# Autodesk Inventor assembly: FinalBioprinter
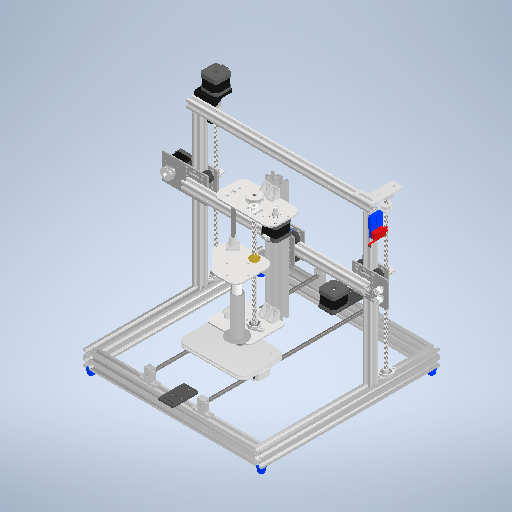
[picture p0: Inventor's stored thumbnail of the model, 512x512]
Saved by Autodesk Inventor 2025.2 (Build 292293000, 293)
## iProperties
Created: 2025-07-17
Part Number: FinalBioprinter
Document SubType Name: Assembly
Designer: Simon
Author: Simon
## Documents named in this file (51)
- C:\Users\Simon\Projects\Hydrogel-3D-Printer\Hardware\Bioprinter Machine Design\Final System\FinalBioprinter.iam
- C:\Users\Simon\Projects\Hydrogel-3D-Printer\Hardware\Bioprinter Machine Design\Final System\Final Gantry\2040_AluminimProfile_410.ipt
- C:\Users\Simon\Projects\Hydrogel-3D-Printer\Hardware\Bioprinter Machine Design\Final System\Final Gantry\2040_AluminimProfile_450.ipt
- C:\Users\Simon\Projects\Hydrogel-3D-Printer\Hardware\Bioprinter Machine Design\Final System\Final Gantry\2020_AluminiumProfile_380.ipt
- C:\Users\Simon\Projects\Hydrogel-3D-Printer\Hardware\Bioprinter Machine Design\Final System\Final Gantry\2020_AluminiumProfile_465.ipt
- C:\Users\Simon\Projects\Hydrogel-3D-Printer\Hardware\Bioprinter Machine Design\PartsFolder\bracket nema 17.ipt
- C:\Users\Simon\Projects\Hydrogel-3D-Printer\Hardware\Bioprinter Machine Design\PartsFolder\Pillow Block Bearing 1\Zinc Alloy Pillow Block Flange Bearing KFL08 ID-8mm.iam
- C:\Users\Simon\Projects\Hydrogel-3D-Printer\Hardware\Bioprinter Machine Design\PartsFolder\Stepper_17HS4401.ipt
- C:\Users\Simon\Projects\Hydrogel-3D-Printer\Hardware\Bioprinter Machine Design\PartsFolder\Flexible Coupling 5,8.ipt
- C:\Users\Simon\Projects\Hydrogel-3D-Printer\Hardware\Bioprinter Machine Design\Final System\Final Gantry\TR8x8-4_LeadScrew_385.ipt
- C:\Users\Simon\Projects\Hydrogel-3D-Printer\Hardware\Bioprinter Machine Design\PartsFolder\TR8x8-4_Nut.ipt
- C:\Users\Simon\Projects\Hydrogel-3D-Printer\Hardware\Bioprinter Machine Design\PartsFolder\Nema 17 Flat Mount.ipt
- C:\Users\Simon\Projects\Hydrogel-3D-Printer\Hardware\Bioprinter Machine Design\PartsFolder\GT2_20T_5.ipt
- C:\Users\Simon\Projects\Hydrogel-3D-Printer\Hardware\Bioprinter Machine Design\PartsFolder\SK8_LinearShaftSupport.ipt
- C:\Users\Simon\Projects\Hydrogel-3D-Printer\Hardware\Bioprinter Machine Design\Final System\Final Gantry\SteelShaft_444mm.ipt
- C:\Users\Simon\Projects\Hydrogel-3D-Printer\Hardware\Bioprinter Machine Design\PartsFolder\SC8UU\SC8UU.iam
- C:\Users\Simon\Projects\Hydrogel-3D-Printer\Hardware\Bioprinter Machine Design\PartsFolder\POM Wheel v2.ipt
- C:\Users\Simon\Projects\Hydrogel-3D-Printer\Hardware\Bioprinter Machine Design\PartsFolder\Carriage Plate v1.ipt
- C:\Users\Simon\Projects\Hydrogel-3D-Printer\Hardware\Bioprinter Machine Design\PartsFolder\Spacer v2.ipt
- C:\Users\Simon\Projects\Hydrogel-3D-Printer\Hardware\Bioprinter Machine Design\Final System\Final Gantry\2020_AluminiumProfile_460.ipt
- C:\Users\Simon\Projects\Hydrogel-3D-Printer\Hardware\Bioprinter Machine Design\Final System\Final Gantry\LeadCarriageConnector.ipt
- C:\Users\Simon\Projects\Hydrogel-3D-Printer\Hardware\Bioprinter Machine Design\Final System\Final Gantry\CarriagePlate_Motor.ipt
- C:\Users\Simon\Projects\Hydrogel-3D-Printer\Hardware\Bioprinter Machine Design\Final System\Final Gantry\CarriagePlate_Idler.ipt
- C:\Users\Simon\Projects\Hydrogel-3D-Printer\Hardware\Bioprinter Machine Design\PartsFolder\GT2_20T_Toothed_Idler_5.ipt
- C:\Users\Simon\Projects\Hydrogel-3D-Printer\Hardware\Bioprinter Machine Design\PartsFolder\Idler Pulley Plate.ipt
- C:\Users\Simon\Projects\Hydrogel-3D-Printer\Hardware\Bioprinter Machine Design\Final System\Final Gantry\BedHeatSink.ipt
- C:\Users\Simon\Projects\Hydrogel-3D-Printer\Hardware\Bioprinter Machine Design\PartsFolder\PeltierTEC1_12706.ipt
- C:\Users\Simon\Projects\Hydrogel-3D-Printer\Hardware\Bioprinter Machine Design\Final System\Final Gantry\ColdPlate.ipt
- C:\Users\Simon\Projects\Hydrogel-3D-Printer\Hardware\Bioprinter Machine Design\Final System\Final Gantry\LeadScrewEndMount.ipt
- C:\Users\Simon\Projects\Hydrogel-3D-Printer\Hardware\Bioprinter Machine Design\PartsFolder\GT2_36T_5.ipt
- C:\Users\Simon\Projects\Hydrogel-3D-Printer\Hardware\Bioprinter Machine Design\PartsFolder\GT2_30T_8.ipt
- C:\Users\Simon\Projects\Hydrogel-3D-Printer\Hardware\Bioprinter Machine Design\Gantry Concept 3\LimitSwitch.ipt
- C:\Users\Simon\Projects\Hydrogel-3D-Printer\Hardware\Bioprinter Machine Design\PartsFolder\Limit Switch\LimitSwitchPart.iam
- C:\Users\Simon\Projects\Hydrogel-3D-Printer\Hardware\Bioprinter Machine Design\Final System\Final Gantry\PrinterFeet.ipt
- C:\Users\Simon\Projects\Hydrogel-3D-Printer\Hardware\Bioprinter Machine Design\PartsFolder\0.4 nozzle.ipt
- C:\Users\Simon\Projects\Hydrogel-3D-Printer\Hardware\Bioprinter Machine Design\PartsFolder\E3D-v6 Heater Block for Sensor Cartridges.ipt
- C:\Users\Simon\Projects\Hydrogel-3D-Printer\Hardware\Bioprinter Machine Design\Final System\Final Extruder\TR8x8-4_LeadScrew_285.ipt
- C:\Users\Simon\Projects\Hydrogel-3D-Printer\Hardware\Bioprinter Machine Design\PartsFolder\GT2_16T_5.ipt
- C:\Users\Simon\Projects\Hydrogel-3D-Printer\Hardware\Bioprinter Machine Design\PartsFolder\GT2_48T_8.ipt
- C:\Users\Simon\Projects\Hydrogel-3D-Printer\Hardware\Bioprinter Machine Design\Final System\Final Extruder\2040_AluminimProfile_x.ipt
- C:\Users\Simon\Projects\Hydrogel-3D-Printer\Hardware\Bioprinter Machine Design\Final System\Final Extruder\Plunger.ipt
- C:\Users\Simon\Projects\Hydrogel-3D-Printer\Hardware\Bioprinter Machine Design\Final System\Final Extruder\CylinderAttachment.ipt
- C:\Users\Simon\Projects\Hydrogel-3D-Printer\Hardware\Bioprinter Machine Design\Final System\Final Extruder\SteelShaft_264.ipt
- C:\Users\Simon\Projects\Hydrogel-3D-Printer\Hardware\Bioprinter Machine Design\PartsFolder\SHF8.ipt
- C:\Users\Simon\Projects\Hydrogel-3D-Printer\Hardware\Bioprinter Machine Design\PartsFolder\LMK8UU.ipt
- C:\Users\Simon\Projects\Hydrogel-3D-Printer\Hardware\Bioprinter Machine Design\Final System\Final Extruder\TopMount.ipt
- C:\Users\Simon\Projects\Hydrogel-3D-Printer\Hardware\Bioprinter Machine Design\Final System\Final Extruder\MidMount.ipt
- C:\Users\Simon\Projects\Hydrogel-3D-Printer\Hardware\Bioprinter Machine Design\Final System\Final Extruder\BottomMount.ipt
- C:\Users\Simon\Projects\Hydrogel-3D-Printer\Hardware\Bioprinter Machine Design\PartsFolder\2020-corner-bracket.ipt
- C:\Users\Simon\Projects\Hydrogel-3D-Printer\Hardware\Bioprinter Machine Design\PartsFolder\GT2_20T_Smooth_Idler_5.ipt
- C:\Users\Simon\Projects\Hydrogel-3D-Printer\Hardware\Bioprinter Machine Design\Final System\Final Extruder\LoadCellMount.ipt
## Components (121 placed, 50 different names)
1. 2040_AluminimProfile_410:1 — Flush:67, Flush:68
2. 2040_AluminimProfile_450:1 — Flush:70, Mate:150
3. 2040_AluminimProfile_410:2 — Flush:70, Mate:151
4. 2040_AluminimProfile_450:2 — Flush:67, Flush:68, Flush:69
5. 2020_AluminiumProfile_380:1
6. 2020_AluminiumProfile_380:2
7. 2020_AluminiumProfile_465:1
8. bracket nema 17:1
9. Zinc Alloy Pillow Block Flange Bearing KFL08 ID-8mm:1 [sub-assembly]
10. Zinc Alloy Pillow Block Flange Bearing KFL08 ID-8mm:2 [sub-assembly]
11. Stepper_17HS4401:1
12. Flexible Coupling 5,8:1
13. TR8x8-4_LeadScrew_385:1
14. TR8x8-4_LeadScrew_385:2
15. TR8x8-4_Nut:1
16. TR8x8-4_Nut:2
17. Nema 17 Flat Mount:1 — Angle:11
18. Stepper_17HS4401:2 — Angle:11
19. GT2_20T_5:1
20. SK8_LinearShaftSupport:1
21. SK8_LinearShaftSupport:2
22. SK8_LinearShaftSupport:3
23. SK8_LinearShaftSupport:4 — Flush:69
24. SteelShaft_444mm:1
25. SteelShaft_444mm:2
26. SC8UU:1 [sub-assembly]
27. SC8UU:2 [sub-assembly]
28. POM Wheel v2:1
29. POM Wheel v2:2
30. POM Wheel v2:3
31. POM Wheel v2:4
32. Carriage Plate v1:1
33. Spacer v2:1
34. Spacer v2:2
35. Spacer v2:3
36. Spacer v2:4
37. Spacer v2:5
38. Spacer v2:6
39. Spacer v2:7
40. Spacer v2:8
41. POM Wheel v2:5
42. POM Wheel v2:6
43. POM Wheel v2:7
44. POM Wheel v2:8
45. Carriage Plate v1:2
46. Spacer v2:9
47. Spacer v2:10
48. Spacer v2:11
49. Spacer v2:12
50. Spacer v2:13
51. Spacer v2:14
52. Spacer v2:15
53. Spacer v2:16
54. 2020_AluminiumProfile_460:1
55. LeadCarriageConnector:1
56. LeadCarriageConnector:2
57. POM Wheel v2:9
58. POM Wheel v2:10
59. POM Wheel v2:11
60. POM Wheel v2:12
61. Carriage Plate v1:3
62. Spacer v2:17
63. Spacer v2:18
64. Spacer v2:19
65. Spacer v2:20
66. Spacer v2:21
67. Spacer v2:22
68. Spacer v2:23
69. Spacer v2:24
70. Carriage Plate v1:4 — Mate:202, Flush:82, Flush:83
71. Stepper_17HS4401:3
72. CarriagePlate_Motor:1
73. CarriagePlate_Idler:1
74. GT2_20T_Toothed_Idler_5:1
75. Spacer v2:25
76. Zinc Alloy Pillow Block Flange Bearing KFL08 ID-8mm:3 [sub-assembly]
77. Idler Pulley Plate:1
78. BedHeatSink:1
79. GT2_20T_Toothed_Idler_5:2
80. PeltierTEC1_12706:1
81. ColdPlate:1
82. Spacer v2:26
83. LeadScrewEndMount:1
84. GT2_20T_Toothed_Idler_5:3
85. Spacer v2:27
86. GT2_36T_5:1
87. GT2_30T_8:1
88. GT2_30T_8:2
89. LimitSwitch:1
90. LimitSwitch:2
91. LimitSwitchPart:1 [sub-assembly]
92. LimitSwitchPart:2 [sub-assembly]
93. PrinterFeet:1
94. PrinterFeet:2 — Mate:149
95. PrinterFeet:3
96. PrinterFeet:4
97. 0.4 nozzle:1
98. E3D-v6 Heater Block for Sensor Cartridges:1
99. TR8x8-4_LeadScrew_285:1
100. Stepper_17HS4401:4
101. TR8x8-4_Nut:3
102. GT2_16T_5:1
103. GT2_48T_8:1
104. Zinc Alloy Pillow Block Flange Bearing KFL08 ID-8mm:4 [sub-assembly]
105. 2040_AluminimProfile_x:1 — Mate:202, Flush:82, Flush:83
106. Plunger:1 — Mate:203
107. CylinderAttachment:1
108. Zinc Alloy Pillow Block Flange Bearing KFL08 ID-8mm:5 [sub-assembly]
109. SteelShaft_264:1
110. SHF8:1
111. SHF8:2
112. LMK8UU:1
113. TopMount:1
114. MidMount:1 — Mate:203
115. BottomMount:1
116. 2020-corner-bracket:1
117. 2020-corner-bracket:2
118. 2020-corner-bracket:3
119. 2020-corner-bracket:4
120. GT2_20T_Smooth_Idler_5:1
121. LoadCellMount:1
## Relationships (299: Mate 201, Flush 83, Angle 15)
- [Mate]: 2040_AluminimProfile_410:1 ↔ 2040_AluminimProfile_450:1
- [Flush]: 2040_AluminimProfile_410:1 ↔ 2040_AluminimProfile_450:1
- [Mate]: 2040_AluminimProfile_450:1 ↔ 2040_AluminimProfile_410:2
- [Flush]: 2040_AluminimProfile_450:1 ↔ 2040_AluminimProfile_410:2
- [Mate]: 2040_AluminimProfile_410:1 ↔ 2040_AluminimProfile_450:2
- [Mate]: 2040_AluminimProfile_450:1 ↔ 2020_AluminiumProfile_380:1
- [Mate]: 2040_AluminimProfile_450:2 ↔ 2020_AluminiumProfile_380:2
- [Flush]: 2040_AluminimProfile_450:1 ↔ 2020_AluminiumProfile_380:1
- [Flush]: 2040_AluminimProfile_450:2 ↔ 2020_AluminiumProfile_380:2
- [Mate]: 2020_AluminiumProfile_380:2 ↔ 2020_AluminiumProfile_465:1
- [Flush]: 2020_AluminiumProfile_380:2 ↔ 2020_AluminiumProfile_465:1
- [Flush]: 2020_AluminiumProfile_380:2 ↔ 2020_AluminiumProfile_465:1
- [Flush]: 2020_AluminiumProfile_380:1 ↔ 2020_AluminiumProfile_465:1
- [Mate]: 2040_AluminimProfile_450:1 ↔ Zinc Alloy Pillow Block Flange Bearing KFL08 ID-8mm:1
- [Mate]: 2040_AluminimProfile_450:2 ↔ Zinc Alloy Pillow Block Flange Bearing KFL08 ID-8mm:2
- [Mate]: 2040_AluminimProfile_450:1 ↔ Zinc Alloy Pillow Block Flange Bearing KFL08 ID-8mm:1
- [Mate]: 2040_AluminimProfile_450:2 ↔ Zinc Alloy Pillow Block Flange Bearing KFL08 ID-8mm:2
- [Flush]: Zinc Alloy Pillow Block Flange Bearing KFL08 ID-8mm:1 ↔ Zinc Alloy Pillow Block Flange Bearing KFL08 ID-8mm:2
- [Mate]: 2020_AluminiumProfile_465:1 ↔ bracket nema 17:1
- [Mate]: bracket nema 17:1 ↔ Zinc Alloy Pillow Block Flange Bearing KFL08 ID-8mm:1
- [Flush] (-10 mm): 2020_AluminiumProfile_465:1 ↔ bracket nema 17:1
- [Mate]: bracket nema 17:1 ↔ Stepper_17HS4401:1
- [Mate]: bracket nema 17:1 ↔ Stepper_17HS4401:1
- [Angle] (0 deg): bracket nema 17:1 ↔ Stepper_17HS4401:1
- [Mate]: Stepper_17HS4401:1 ↔ Flexible Coupling 5,8:1
- [Flush] (5 mm): Stepper_17HS4401:1 ↔ Flexible Coupling 5,8:1
- [Mate]: Zinc Alloy Pillow Block Flange Bearing KFL08 ID-8mm:1 ↔ TR8x8-4_LeadScrew_385:1
- [Mate]: Zinc Alloy Pillow Block Flange Bearing KFL08 ID-8mm:2 ↔ TR8x8-4_LeadScrew_385:2
- [Flush]: TR8x8-4_LeadScrew_385:1 ↔ TR8x8-4_LeadScrew_385:2
- [Mate]: Stepper_17HS4401:1 ↔ TR8x8-4_LeadScrew_385:1
- [Mate]: TR8x8-4_LeadScrew_385:1 ↔ TR8x8-4_Nut:1
- [Mate]: TR8x8-4_LeadScrew_385:2 ↔ TR8x8-4_Nut:2
- [Flush]: TR8x8-4_Nut:1 ↔ TR8x8-4_Nut:2
- [Mate]: 2040_AluminimProfile_410:2 ↔ Nema 17 Flat Mount:1
- [Mate]: 2040_AluminimProfile_410:2 ↔ Nema 17 Flat Mount:1
- [Mate]: Nema 17 Flat Mount:1 ↔ Stepper_17HS4401:2
- [Mate]: Nema 17 Flat Mount:1 ↔ Stepper_17HS4401:2
- [Mate]: Stepper_17HS4401:2 ↔ GT2_20T_5:1
- [Mate]: 2040_AluminimProfile_410:2 ↔ SK8_LinearShaftSupport:1
- [Mate]: 2040_AluminimProfile_410:2 ↔ SK8_LinearShaftSupport:2
- [Mate]: 2040_AluminimProfile_410:1 ↔ SK8_LinearShaftSupport:3
- [Mate]: 2040_AluminimProfile_410:1 ↔ SK8_LinearShaftSupport:4
- [Flush]: 2040_AluminimProfile_410:2 ↔ SK8_LinearShaftSupport:1
- [Flush]: 2040_AluminimProfile_410:2 ↔ SK8_LinearShaftSupport:2
- [Flush]: 2040_AluminimProfile_410:1 ↔ SK8_LinearShaftSupport:4
- [Flush]: 2040_AluminimProfile_410:1 ↔ SK8_LinearShaftSupport:3
- [Mate]: SK8_LinearShaftSupport:1 ↔ SK8_LinearShaftSupport:3
- [Mate]: SK8_LinearShaftSupport:2 ↔ SK8_LinearShaftSupport:4
- [Mate]: SK8_LinearShaftSupport:3 ↔ SteelShaft_444mm:1
- [Mate]: SK8_LinearShaftSupport:4 ↔ SteelShaft_444mm:2
- [Flush]: SK8_LinearShaftSupport:3 ↔ SteelShaft_444mm:1
- [Flush]: SK8_LinearShaftSupport:4 ↔ SteelShaft_444mm:2
- [Mate]: SteelShaft_444mm:1 ↔ SC8UU:1
- [Mate]: SteelShaft_444mm:2 ↔ SC8UU:2
- [Angle] (0 deg): 2040_AluminimProfile_450:1 ↔ SC8UU:1
- [Angle] (0 deg): 2040_AluminimProfile_450:2 ↔ SC8UU:2
- [Flush]: SC8UU:1 ↔ SC8UU:2
- [Mate]: POM Wheel v2:1 ↔ Carriage Plate v1:1
- [Mate]: Carriage Plate v1:1 ↔ Spacer v2:5
- [Mate]: Carriage Plate v1:1 ↔ Spacer v2:6
- [Mate]: Carriage Plate v1:1 ↔ Spacer v2:7
- [Mate]: Carriage Plate v1:1 ↔ Spacer v2:8
- [Flush]: Spacer v2:5 ↔ Spacer v2:6
- [Flush]: Spacer v2:6 ↔ Spacer v2:7
- [Flush]: Spacer v2:7 ↔ Spacer v2:8
- [Mate]: Carriage Plate v1:1 ↔ Spacer v2:6
- [Flush]: Spacer v2:1 ↔ Spacer v2:2
- [Flush]: Spacer v2:2 ↔ Spacer v2:3
- [Flush]: Spacer v2:3 ↔ Spacer v2:4
- [Flush]: POM Wheel v2:1 ↔ POM Wheel v2:2
- [Flush]: POM Wheel v2:2 ↔ POM Wheel v2:3
- [Flush]: POM Wheel v2:3 ↔ POM Wheel v2:4
- [Mate]: POM Wheel v2:2 ↔ Spacer v2:6
- [Mate]: POM Wheel v2:1 ↔ Spacer v2:1
- [Mate]: POM Wheel v2:5 ↔ Carriage Plate v1:2
- [Mate]: Carriage Plate v1:2 ↔ Spacer v2:13
- [Mate]: Carriage Plate v1:2 ↔ Spacer v2:14
- [Mate]: Carriage Plate v1:2 ↔ Spacer v2:15
- [Mate]: Carriage Plate v1:2 ↔ Spacer v2:16
- [Flush]: Spacer v2:13 ↔ Spacer v2:14
- [Flush]: Spacer v2:14 ↔ Spacer v2:15
- [Flush]: Spacer v2:15 ↔ Spacer v2:16
- [Mate]: Carriage Plate v1:2 ↔ Spacer v2:14
- [Flush]: Spacer v2:9 ↔ Spacer v2:10
- [Flush]: Spacer v2:10 ↔ Spacer v2:11
- [Flush]: Spacer v2:11 ↔ Spacer v2:12
- [Flush]: POM Wheel v2:5 ↔ POM Wheel v2:6
- [Flush]: POM Wheel v2:6 ↔ POM Wheel v2:7
- [Flush]: POM Wheel v2:7 ↔ POM Wheel v2:8
- [Mate]: POM Wheel v2:6 ↔ Spacer v2:14
- [Mate]: POM Wheel v2:5 ↔ Spacer v2:9
- [Mate]: 2020_AluminiumProfile_380:1 ↔ POM Wheel v2:2
- [Mate]: 2020_AluminiumProfile_380:2 ↔ POM Wheel v2:6
- [Mate]: Carriage Plate v1:2 ↔ LeadCarriageConnector:1
- [Mate]: Carriage Plate v1:1 ↔ LeadCarriageConnector:2
- [Mate]: Carriage Plate v1:2 ↔ LeadCarriageConnector:1
- [Mate]: Carriage Plate v1:1 ↔ LeadCarriageConnector:2
- [Mate]: Carriage Plate v1:2 ↔ LeadCarriageConnector:1
- [Mate]: Carriage Plate v1:1 ↔ LeadCarriageConnector:2
- [Angle] (0 deg): TR8x8-4_Nut:2 ↔ LeadCarriageConnector:1
- [Angle] (0 deg): TR8x8-4_Nut:1 ↔ LeadCarriageConnector:2
- [Mate]: TR8x8-4_Nut:1 ↔ LeadCarriageConnector:2
- [Mate]: POM Wheel v2:5 ↔ Spacer v2:9
- [Mate]: Spacer v2:12 ↔ Spacer v2:16
- [Mate]: Spacer v2:10 ↔ Spacer v2:14
- [Mate]: Spacer v2:11 ↔ Spacer v2:15
- [Mate]: POM Wheel v2:7 ↔ Spacer v2:11
- [Mate]: POM Wheel v2:8 ↔ Spacer v2:16
- [Mate]: POM Wheel v2:6 ↔ Spacer v2:14
- [Mate]: 2020_AluminiumProfile_380:2 ↔ Carriage Plate v1:2
- [Flush]: Carriage Plate v1:1 ↔ Carriage Plate v1:2
- [Mate]: POM Wheel v2:1 ↔ Spacer v2:1
- [Mate]: Spacer v2:2 ↔ Spacer v2:6
- [Mate]: Spacer v2:4 ↔ Spacer v2:8
- [Mate]: Spacer v2:3 ↔ Spacer v2:7
- [Mate]: POM Wheel v2:4 ↔ Spacer v2:8
- [Mate]: POM Wheel v2:3 ↔ Spacer v2:7
- [Mate]: POM Wheel v2:2 ↔ Spacer v2:2
- [Flush]: 2020_AluminiumProfile_380:1 ↔ Carriage Plate v1:1
- [Mate]: POM Wheel v2:9 ↔ Carriage Plate v1:3
- [Mate]: Carriage Plate v1:3 ↔ Spacer v2:21
- [Mate]: Carriage Plate v1:3 ↔ Spacer v2:22
- [Mate]: Carriage Plate v1:3 ↔ Spacer v2:23
- [Mate]: Carriage Plate v1:3 ↔ Spacer v2:24
- [Flush]: Spacer v2:21 ↔ Spacer v2:22
- [Flush]: Spacer v2:22 ↔ Spacer v2:23
- [Flush]: Spacer v2:23 ↔ Spacer v2:24
- [Mate]: Carriage Plate v1:3 ↔ Spacer v2:22
- [Flush]: Spacer v2:17 ↔ Spacer v2:18
- [Flush]: Spacer v2:18 ↔ Spacer v2:19
- [Flush]: Spacer v2:19 ↔ Spacer v2:20
- [Flush]: POM Wheel v2:9 ↔ POM Wheel v2:10
- [Flush]: POM Wheel v2:10 ↔ POM Wheel v2:11
- [Flush]: POM Wheel v2:11 ↔ POM Wheel v2:12
- [Mate]: POM Wheel v2:10 ↔ Spacer v2:22
- [Mate]: POM Wheel v2:9 ↔ Spacer v2:17
- [Mate]: POM Wheel v2:9 ↔ Spacer v2:17
- [Mate]: Spacer v2:18 ↔ Spacer v2:22
- [Mate]: Spacer v2:20 ↔ Spacer v2:24
- [Mate]: Spacer v2:19 ↔ Spacer v2:23
- [Mate]: POM Wheel v2:12 ↔ Spacer v2:24
- [Mate]: POM Wheel v2:11 ↔ Spacer v2:23
- [Mate]: POM Wheel v2:10 ↔ Spacer v2:18
- [Flush] (225 mm): 2040_AluminimProfile_450:2 ↔ 2020_AluminiumProfile_460:1
- [Flush]: 2020_AluminiumProfile_460:1 ↔ POM Wheel v2:9
- [Flush]: 2020_AluminiumProfile_460:1 ↔ Carriage Plate v1:3
- [Mate]: Spacer v2:19 ↔ Carriage Plate v1:4
- [Mate]: Spacer v2:17 ↔ Carriage Plate v1:4
- [Mate]: Spacer v2:18 ↔ Carriage Plate v1:4
- [Mate]: Spacer v2:4 ↔ CarriagePlate_Motor:1
- [Mate]: Spacer v2:2 ↔ CarriagePlate_Motor:1
- [Mate]: Spacer v2:4 ↔ CarriagePlate_Motor:1
- [Mate]: 2020_AluminiumProfile_460:1 ↔ CarriagePlate_Motor:1
- [Flush]: 2020_AluminiumProfile_460:1 ↔ CarriagePlate_Motor:1
- [Mate]: Stepper_17HS4401:3 ↔ CarriagePlate_Motor:1
- [Mate]: Stepper_17HS4401:3 ↔ CarriagePlate_Motor:1
- [Angle] (0 deg): Stepper_17HS4401:3 ↔ CarriagePlate_Motor:1
- [Mate]: Spacer v2:11 ↔ CarriagePlate_Idler:1
- [Mate]: Spacer v2:9 ↔ CarriagePlate_Idler:1
- [Mate]: Spacer v2:10 ↔ CarriagePlate_Idler:1
- [Mate]: CarriagePlate_Idler:1 ↔ Spacer v2:25
- [Mate]: GT2_20T_Toothed_Idler_5:1 ↔ Spacer v2:25
- [Flush] (275 mm): 2040_AluminimProfile_410:1 ↔ 2020_AluminiumProfile_380:2
- [Mate]: TR8x8-4_LeadScrew_385:2 ↔ Zinc Alloy Pillow Block Flange Bearing KFL08 ID-8mm:3
- [Flush]: 2020_AluminiumProfile_465:1 ↔ Zinc Alloy Pillow Block Flange Bearing KFL08 ID-8mm:3
- [Mate]: Zinc Alloy Pillow Block Flange Bearing KFL08 ID-8mm:2 ↔ Zinc Alloy Pillow Block Flange Bearing KFL08 ID-8mm:3
- [Mate]: 2040_AluminimProfile_410:1 ↔ Idler Pulley Plate:1
- [Flush]: Nema 17 Flat Mount:1 ↔ Idler Pulley Plate:1
- [Mate]: SC8UU:1 ↔ BedHeatSink:1
- [Mate]: SC8UU:2 ↔ BedHeatSink:1
- [Mate]: SC8UU:2 ↔ BedHeatSink:1
- [Flush]: 2040_AluminimProfile_410:1 ↔ Idler Pulley Plate:1
- [Mate]: 2040_AluminimProfile_410:1 ↔ Idler Pulley Plate:1
- [Mate]: Idler Pulley Plate:1 ↔ GT2_20T_Toothed_Idler_5:2
- [Flush]: GT2_20T_5:1 ↔ GT2_20T_Toothed_Idler_5:2
- [Mate]: BedHeatSink:1 ↔ PeltierTEC1_12706:1
- [Angle] (0 deg): BedHeatSink:1 ↔ PeltierTEC1_12706:1
- [Mate]: BedHeatSink:1 ↔ PeltierTEC1_12706:1
- [Flush]: BedHeatSink:1 ↔ PeltierTEC1_12706:1
- [Mate]: BedHeatSink:1 ↔ ColdPlate:1
- [Mate]: BedHeatSink:1 ↔ ColdPlate:1
- [Mate]: PeltierTEC1_12706:1 ↔ ColdPlate:1
- [Mate]: Idler Pulley Plate:1 ↔ Spacer v2:26
- [Mate]: Idler Pulley Plate:1 ↔ Spacer v2:26
- [Mate]: GT2_20T_Toothed_Idler_5:2 ↔ Spacer v2:26
- [Mate]: 2020_AluminiumProfile_465:1 ↔ LeadScrewEndMount:1
- [Flush]: 2020_AluminiumProfile_465:1 ↔ LeadScrewEndMount:1
- [Flush] (-4 mm): 2020_AluminiumProfile_465:1 ↔ LeadScrewEndMount:1
- [Mate]: CarriagePlate_Idler:1 ↔ Spacer v2:25
- [Mate]: GT2_20T_Toothed_Idler_5:1 ↔ Spacer v2:25
- [Mate]: GT2_20T_Toothed_Idler_5:3 ↔ Spacer v2:27
- [Mate]: GT2_20T_Toothed_Idler_5:3 ↔ Spacer v2:27
- [Mate]: CarriagePlate_Idler:1 ↔ Spacer v2:27
- [Mate]: CarriagePlate_Idler:1 ↔ GT2_20T_Toothed_Idler_5:3
- [Mate]: Stepper_17HS4401:3 ↔ GT2_36T_5:1
- [Flush]: GT2_20T_Toothed_Idler_5:1 ↔ GT2_36T_5:1
- [Mate]: TR8x8-4_LeadScrew_385:2 ↔ GT2_30T_8:2
- [Mate]: TR8x8-4_LeadScrew_385:1 ↔ GT2_30T_8:1
- [Flush]: GT2_30T_8:1 ↔ GT2_30T_8:2
- [Mate]: Flexible Coupling 5,8:1 ↔ GT2_30T_8:1
- [Mate]: 2020_AluminiumProfile_380:2 ↔ LimitSwitch:1
- [Mate]: Carriage Plate v1:3 ↔ LimitSwitch:2
- [Angle] (0 deg): Carriage Plate v1:3 ↔ LimitSwitch:2
- [Mate]: Carriage Plate v1:3 ↔ LimitSwitch:2
- [Mate]: LimitSwitch:2 ↔ LimitSwitchPart:2
- [Angle] (0 deg): LimitSwitch:2 ↔ LimitSwitchPart:2
- [Mate]: LimitSwitch:2 ↔ LimitSwitchPart:2
- [Flush]: 2020_AluminiumProfile_380:2 ↔ LimitSwitch:1
- [Mate] (20 mm): LeadScrewEndMount:1 ↔ LimitSwitch:1
- [Mate]: LimitSwitch:1 ↔ LimitSwitchPart:1
- [Angle] (0 deg): LimitSwitch:1 ↔ LimitSwitchPart:1
- [Mate]: LimitSwitch:1 ↔ LimitSwitchPart:1
- [Flush]: PrinterFeet:2 ↔ PrinterFeet:3
- [Flush]: PrinterFeet:1 ↔ PrinterFeet:2
- [Flush]: PrinterFeet:3 ↔ PrinterFeet:4
- [Mate]: 2040_AluminimProfile_410:1 ↔ PrinterFeet:4
- [Mate]: 2040_AluminimProfile_450:2 ↔ PrinterFeet:4
- [Mate]: 2040_AluminimProfile_450:2 ↔ PrinterFeet:3
- [Mate]: 2040_AluminimProfile_410:2 ↔ PrinterFeet:3
- [Mate]: 2040_AluminimProfile_450:1 ↔ PrinterFeet:1
- [Mate]: 2040_AluminimProfile_410:2 ↔ PrinterFeet:1
- [Mate]: 2040_AluminimProfile_410:1 ↔ PrinterFeet:2
- [Mate]: 2040_AluminimProfile_450:1 ↔ PrinterFeet:2
- [Mate]: 2040_AluminimProfile_450:2 ↔ PrinterFeet:4
- Flush:67: 2040_AluminimProfile_410:1 ↔ 2040_AluminimProfile_450:2
- Flush:68: 2040_AluminimProfile_410:1 ↔ 2040_AluminimProfile_450:2
- Flush:69 (137 mm): 2040_AluminimProfile_450:2 ↔ SK8_LinearShaftSupport:4
- Flush:70: 2040_AluminimProfile_450:1 ↔ 2040_AluminimProfile_410:2
- Mate:149: PrinterFeet:2
- Mate:150: 2040_AluminimProfile_450:1
- Mate:151: 2040_AluminimProfile_410:2
- Angle:11 (0 deg): Nema 17 Flat Mount:1 ↔ Stepper_17HS4401:2
- [Mate]: 0.4 nozzle:1 ↔ E3D-v6 Heater Block for Sensor Cartridges:1
- [Mate]: 0.4 nozzle:1 ↔ E3D-v6 Heater Block for Sensor Cartridges:1
- [Angle] (0 deg): 0.4 nozzle:1 ↔ E3D-v6 Heater Block for Sensor Cartridges:1
- [Mate]: TR8x8-4_LeadScrew_285:1 ↔ TR8x8-4_Nut:3
- [Mate]: TR8x8-4_LeadScrew_285:1 ↔ GT2_48T_8:1
- [Mate]: Stepper_17HS4401:4 ↔ GT2_16T_5:1
- [Mate]: TR8x8-4_LeadScrew_285:1 ↔ Zinc Alloy Pillow Block Flange Bearing KFL08 ID-8mm:4
- [Mate]: E3D-v6 Heater Block for Sensor Cartridges:1 ↔ CylinderAttachment:1
- [Mate]: 0.4 nozzle:1 ↔ CylinderAttachment:1
- [Flush]: TR8x8-4_LeadScrew_285:1 ↔ Zinc Alloy Pillow Block Flange Bearing KFL08 ID-8mm:4
- [Mate]: TR8x8-4_LeadScrew_285:1 ↔ Zinc Alloy Pillow Block Flange Bearing KFL08 ID-8mm:5
- [Mate]: SteelShaft_264:1 ↔ SHF8:1
- [Mate]: SteelShaft_264:1 ↔ SHF8:2
- [Flush]: SteelShaft_264:1 ↔ SHF8:1
- [Flush]: SteelShaft_264:1 ↔ SHF8:2
- [Flush]: 2040_AluminimProfile_x:1 ↔ TopMount:1
- [Mate]: 2040_AluminimProfile_x:1 ↔ TopMount:1
- [Flush]: 2040_AluminimProfile_x:1 ↔ BottomMount:1
- [Mate]: 2040_AluminimProfile_x:1 ↔ BottomMount:1
- [Mate]: Stepper_17HS4401:4 ↔ TopMount:1
- [Angle] (90 deg): Stepper_17HS4401:4 ↔ TopMount:1
- [Flush]: Stepper_17HS4401:4 ↔ GT2_16T_5:1
- [Mate]: SHF8:2 ↔ TopMount:1
- [Mate]: Zinc Alloy Pillow Block Flange Bearing KFL08 ID-8mm:5 ↔ TopMount:1
- [Mate]: CylinderAttachment:1 ↔ BottomMount:1
- [Flush]: GT2_16T_5:1 ↔ GT2_48T_8:1
- [Mate]: 2040_AluminimProfile_x:1 ↔ 2020-corner-bracket:1
- [Mate]: TopMount:1 ↔ 2020-corner-bracket:1
- [Mate]: 2040_AluminimProfile_x:1 ↔ 2020-corner-bracket:2
- [Mate]: TopMount:1 ↔ 2020-corner-bracket:2
- [Mate]: 2040_AluminimProfile_x:1 ↔ 2020-corner-bracket:3
- [Mate]: BottomMount:1 ↔ 2020-corner-bracket:3
- [Mate]: 2040_AluminimProfile_x:1 ↔ 2020-corner-bracket:4
- [Mate]: BottomMount:1 ↔ 2020-corner-bracket:4
- [Mate]: SteelShaft_264:1 ↔ LMK8UU:1
- [Mate]: Zinc Alloy Pillow Block Flange Bearing KFL08 ID-8mm:4 ↔ BottomMount:1
- [Flush]: 2040_AluminimProfile_x:1 ↔ BottomMount:1
- [Mate]: TR8x8-4_Nut:3 ↔ MidMount:1
- [Mate]: LMK8UU:1 ↔ MidMount:1
- [Mate]: 2040_AluminimProfile_x:1 ↔ 2020-corner-bracket:1
- [Mate]: 2040_AluminimProfile_x:1 ↔ 2020-corner-bracket:2
- [Flush]: 2040_AluminimProfile_x:1 ↔ 2020-corner-bracket:4
- [Mate]: 2040_AluminimProfile_x:1 ↔ 2020-corner-bracket:3
- [Flush] (-10 mm): 2040_AluminimProfile_x:1 ↔ 2020-corner-bracket:2
- [Mate]: Stepper_17HS4401:4 ↔ TopMount:1
- [Mate]: Zinc Alloy Pillow Block Flange Bearing KFL08 ID-8mm:5 ↔ TopMount:1
- [Mate]: SteelShaft_264:1 ↔ TopMount:1
- [Mate]: SHF8:2 ↔ TopMount:1
- [Angle] (0 deg): Zinc Alloy Pillow Block Flange Bearing KFL08 ID-8mm:5 ↔ TopMount:1
- [Mate]: SHF8:1 ↔ BottomMount:1
- [Angle] (0 deg): Zinc Alloy Pillow Block Flange Bearing KFL08 ID-8mm:4 ↔ BottomMount:1
- [Mate]: CylinderAttachment:1 ↔ BottomMount:1
- [Mate]: CylinderAttachment:1 ↔ BottomMount:1
- [Mate]: SteelShaft_264:1 ↔ MidMount:1
- [Mate]: TR8x8-4_Nut:3 ↔ MidMount:1
- [Mate]: LMK8UU:1 ↔ MidMount:1
- [Mate]: TR8x8-4_Nut:3 ↔ MidMount:1
- [Mate]: TopMount:1 ↔ GT2_20T_Smooth_Idler_5:1
- [Flush]: GT2_48T_8:1 ↔ GT2_20T_Smooth_Idler_5:1
- [Mate]: Plunger:1 ↔ CylinderAttachment:1
- [Mate]: Plunger:1 ↔ LoadCellMount:1
- [Mate]: MidMount:1 ↔ LoadCellMount:1
- [Mate]: MidMount:1 ↔ LoadCellMount:1
- Mate:202: Carriage Plate v1:4 ↔ 2040_AluminimProfile_x:1
- Mate:203: Plunger:1 ↔ MidMount:1
- Flush:82 (-120 mm): Carriage Plate v1:4 ↔ 2040_AluminimProfile_x:1
- Flush:83 (12.75 mm): Carriage Plate v1:4 ↔ 2040_AluminimProfile_x:1
## Named parameters: d229_d265 = 0 mm, d230_d266 = 0 mm, d231_d267 = 0 deg, d232_d268 = 0 mm, d233_d269 = 0 mm, d234_d270 = 20 mm, d235_d271 = 0 mm, d238_d206 = 0 mm, d239_d237 = 0 mm, d157_d76 = 0 mm, d158_d78 = 0 mm, d159_d79 = 0 mm, d160_d80 = 0 mm, d161_d81 = 0 mm, d162_d82 = 0 mm, d163_d83 = 0 mm, d164_d84 = 0 mm, d165_d85 = 0 mm, d166_d86 = 0 mm, d167_d87 = 0 mm, d168_d88 = 0 mm, d169_d89 = 0 mm, d170_d90 = 0 mm, d171_d91 = 0 mm, d172_d92 = 0 mm, d173_d93 = 0 mm, d174_d145 = 0 mm, d175_d146 = 0 mm, d176_d147 = 0 mm, d177_d148 = 0 mm, d178_d149 = 0 mm, d179_d150 = 0 mm, d180_d151 = 0 mm, d95_d80 = 0 mm, d96_d81 = 0 mm, d97_d82 = 0 mm, d98_d83 = 0 mm, d99_d84 = 0 mm, d100_d85 = 0 mm, d101_d86 = 0 mm, d102_d87 = 0 mm, d103_d88 = 0 mm, d104_d89 = 0 mm, d105_d90 = 0 mm, d106_d91 = 0 mm, d107_d92 = 0 mm, d108_d93 = 0 mm, d118_d76 = 0 mm, d120_d78 = 0 mm, d121_d79 = 0 mm, d470_d57 = 0 mm, d471_d58 = 0 mm, d472_d59 = 0 mm, d473_d60 = 0 mm, d474_d65 = 0 mm, d475_d66 = 0 mm, d476_d67 = 0 mm, d485_d76 = 0 mm, d487_d78 = -10 mm, d488_d79 = 0 mm, d489_d80 = 0 mm, d490_d81 = 0 mm, d491_d82 = 0 mm, d492_d83 = 0 deg, d493_d84 = 0 mm, d494_d85 = 0 deg, d495_d86 = 0 mm, d496_d87 = 0 mm, d497_d89 = 0 mm, d498_d90 = 0 mm, d499_d93 = 0 mm, d500_d10 = 0 mm, d501_d11 = 0 mm, d502_d32 = 0 mm, d503_d33 = 0 mm, d504_d36 = 0 mm, d505_d38 = 0 mm, d506_d39 = 0 mm, d511_d44 = 0 mm, d512_d47 = 0 mm, d513_d48 = 0 mm, d514_d50 = 0 mm, d515_d51 = 90 deg, d516_d52 = 0 mm, d517_d53 = 0 mm, d518_d54 = 0 mm, d519_d55 = 0 mm, d520_d56 = 0 mm, d524_d7 = 0 mm, d525_d9 = 0 mm
